# Autodesk Inventor assembly: E004_BoitierDeProtection
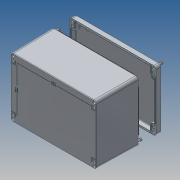
[picture p0: Inventor's stored thumbnail of the model, 180x180]
Saved by Autodesk Inventor 2021.3 (Build 253353000, 353)
## iProperties
Created: 2021-11-18
Part Number: E004_BoitierDeProtection
Document SubType Name: Assembly
Designer: gabri
Author: gabri
## Documents named in this file (3)
- D:\PGA\E004_BoitierDeProtection.iam
- D:\PGA\Boitier_Phoenix_A150.iam
- D:\PGA\P031_MonoVitreBas.ipt
## Components (2 placed, 2 different names)
1. Boitier_Phoenix_A150:1 [sub-assembly] — Flush:1, Mate:1, Mate:2
2. P031_MonoVitreBas:1 — Flush:1, Mate:1, Mate:2
## Relationships (3: Mate 2, Flush 1)
- Flush:1: Boitier_Phoenix_A150:1 ↔ P031_MonoVitreBas:1
- Mate:1: Boitier_Phoenix_A150:1 ↔ P031_MonoVitreBas:1
- Mate:2: Boitier_Phoenix_A150:1 ↔ P031_MonoVitreBas:1
